# Autodesk Inventor assembly: Zonnepaneel 4.0
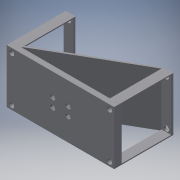
[picture p0: Inventor's stored thumbnail of the model, 180x180]
Saved by Autodesk Inventor 2018.3 (Build 223284000, 284)
## iProperties
Created: 2020-11-23
Part Number: Zonnepaneel 4.0
Document SubType Name: Assembly
Designer: daanv
Author: daanv
## Documents named in this file (4)
- C:\Users\daanv\OneDrive\Documenten\Life\Avans Project RED\Token\Zonnepaneel\V3.0\Zonnepaneel 4.0.iam
- C:\Users\daanv\OneDrive\Documenten\Life\Avans Project RED\Token\Zonnepaneel\V3.0\Hoofdplaat onderkant.ipt
- C:\Users\daanv\OneDrive\Documenten\Life\Avans Project RED\Token\Zonnepaneel\V3.0\Hoofdplaat zijkant.ipt
- C:\Users\daanv\OneDrive\Documenten\Life\Avans Project RED\Token\Zonnepaneel\V3.0\Zonnecel.ipt
## Components (4 placed, 3 different names)
1. Hoofdplaat onderkant:1 — Mate:1, Mate:2, Mate:3, Mate:4
2. Hoofdplaat zijkant:1 — Mate:3, Mate:4, Mate:5, Mate:6
3. Hoofdplaat zijkant:2 — Mate:1, Mate:2
4. Zonnecel:1 — Mate:5, Mate:6
## Relationships (6: Mate 6)
- Mate:1: Hoofdplaat onderkant:1 ↔ Hoofdplaat zijkant:2
- Mate:2: Hoofdplaat onderkant:1 ↔ Hoofdplaat zijkant:2
- Mate:3: Hoofdplaat onderkant:1 ↔ Hoofdplaat zijkant:1
- Mate:4: Hoofdplaat onderkant:1 ↔ Hoofdplaat zijkant:1
- Mate:5: Hoofdplaat zijkant:1 ↔ Zonnecel:1
- Mate:6: Hoofdplaat zijkant:1 ↔ Zonnecel:1
